# Autodesk Inventor assembly: Swingarm2
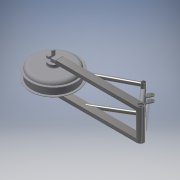
[picture p0: Inventor's stored thumbnail of the model, 180x180]
Saved by Autodesk Inventor 2019.2 (Build 232265000, 265)
## iProperties
Created: 2018-06-07
Part Number: Swingarm2
Document SubType Name: Assembly
Designer: eroldan
Author: eroldan
## Documents named in this file (4)
- C:\Users\eroldan\Desktop\3dprojects\OpenEmoto\Swingarm2\Swingarm2.iam
- C:\Users\eroldan\Desktop\3dprojects\OpenEmoto\OtherParts\HubMotor3KW.ipt
- C:\Users\eroldan\Desktop\3dprojects\OpenEmoto\Swingarm2\Swingarm2.ipt
- C:\Users\eroldan\Desktop\3dprojects\OpenEmoto\Swingarm2\Skirt.ipt
## Components (3 placed, 3 different names)
1. HubMotor3KW:1 — Mate:1, Mate:2, Mate:3
2. Swingarm2:1 — Mate:1, Mate:2, Mate:3, Mate:4, Mate:5
3. Skirt:1 — Flush:1
## Relationships (8: Mate 7, Flush 1)
- Mate:1: HubMotor3KW:1 ↔ Swingarm2:1
- Mate:2: HubMotor3KW:1 ↔ Swingarm2:1
- Mate:3: HubMotor3KW:1 ↔ Swingarm2:1
- Mate:4: Swingarm2:1
- Mate:5: Swingarm2:1
- Mate:6
- Mate:7
- Flush:1: Skirt:1
